# Autodesk Inventor assembly: coxa kiri
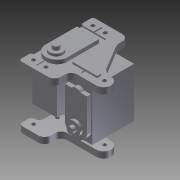
[picture p0: Inventor's stored thumbnail of the model, 180x180]
Saved by Autodesk Inventor 2012 (Build 160160000, 160)
## iProperties
Created: 2013-12-07
Part Number: coxa kiri
Document SubType Name: Assembly
Designer: Irwan Haryanto
Author: Irwan Haryanto
## Documents named in this file (4)
- D:\Revenant\robot baru 2014\coxa kiri.iam
- D:\Revenant\robot baru 2014\braket atas.ipt
- D:\Revenant\robot baru 2014\braket bawah.ipt
- D:\Revenant\robot baru 2014\servo HS-7955GT.ipt
## Components (4 placed, 3 different names)
1. braket atas:1 — Mate:1, Mate:2, Mate:3, Insert:1, Insert:2
2. servo HS-7955GT:1 — Mate:1, Mate:2, Mate:3, Mate:4, Mate:5, Mate:6
3. servo HS-7955GT:2 — Insert:1, Insert:2
4. braket bawah:1 — Mate:4, Mate:5, Mate:6
## Relationships (8: Mate 6, Insert 2)
- Mate:1: braket atas:1 ↔ servo HS-7955GT:1
- Mate:2: braket atas:1 ↔ servo HS-7955GT:1
- Mate:3: braket atas:1 ↔ servo HS-7955GT:1
- Mate:4: servo HS-7955GT:1 ↔ braket bawah:1
- Mate:5: servo HS-7955GT:1 ↔ braket bawah:1
- Mate:6: servo HS-7955GT:1 ↔ braket bawah:1
- Insert:1: braket atas:1 ↔ servo HS-7955GT:2
- Insert:2: braket atas:1 ↔ servo HS-7955GT:2
